# Autodesk Inventor assembly: SensorAssembly
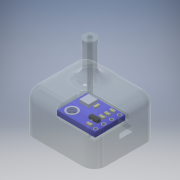
[picture p0: Inventor's stored thumbnail of the model, 180x180]
Saved by Autodesk Inventor 2018 (Build 220112000, 112)
## iProperties
Created: 2020-03-09
Part Number: SensorAssembly
Document SubType Name: Assembly
Designer: Ivan
Author: Ivan
## Documents named in this file (3)
- C:\Users\Ivan\Documents\GitHub\IdealGas\3D Model\SensorAssembly.iam
- C:\Users\Ivan\Documents\GitHub\IdealGas\3D Model\BMP180.ipt
- C:\Users\Ivan\Documents\GitHub\IdealGas\3D Model\DAQcapsule.ipt
## Components (2 placed, 2 different names)
1. BMP180:1 — Mate:1, Mate:2, Angle:1
2. DAQcapsule:1 — Mate:1, Mate:2, Angle:1
## Relationships (3: Mate 2, Angle 1)
- Mate:1: BMP180:1 ↔ DAQcapsule:1
- Mate:2: BMP180:1 ↔ DAQcapsule:1
- Angle:1 (0 deg): BMP180:1 ↔ DAQcapsule:1
